# Autodesk Inventor assembly: POM_T5_06
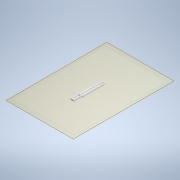
[picture p0: Inventor's stored thumbnail of the model, 180x180]
Saved by Autodesk Inventor 2022 (Build 260153000, 153)
## iProperties
Created: 2022-09-28
Part Number: POM_T5_06
Document SubType Name: Assembly
Designer: Masato
Author: Masato
## Documents named in this file (4)
- C:\Users\6343y\ドキュメント\Inventor\SUSTAINA-OP\Cam\POM_T5\POM_T5_06.iam
- C:\Users\6343y\ドキュメント\Inventor\SUSTAINA-OP\Cam\DisposableBoard.ipt
- C:\Users\6343y\ドキュメント\Inventor\SUSTAINA-OP\OptionParts\DrillingJigs\Cockpit_back_frame_Jig.ipt
- C:\Users\6343y\ドキュメント\Inventor\SUSTAINA-OP\OptionParts\DrillingJigs\Cockpit_front_frame_Jig.ipt
## Components (3 placed, 3 different names)
1. DisposableBoard:1 — フラッシュ:1, フラッシュ:2, フラッシュ:3, フラッシュ:4
2. Cockpit_back_frame_Jig:1 — メイト:1
3. Cockpit_front_frame_Jig:1 — メイト:2
## Relationships (6: Flush 4, Mate 2)
- フラッシュ:1 [Flush]: DisposableBoard:1
- フラッシュ:2 [Flush]: DisposableBoard:1
- フラッシュ:3 [Flush]: DisposableBoard:1
- フラッシュ:4 [Flush]: DisposableBoard:1
- メイト:1 [Mate]: Cockpit_back_frame_Jig:1
- メイト:2 [Mate]: Cockpit_front_frame_Jig:1
